# Autodesk Inventor assembly: maze_version2
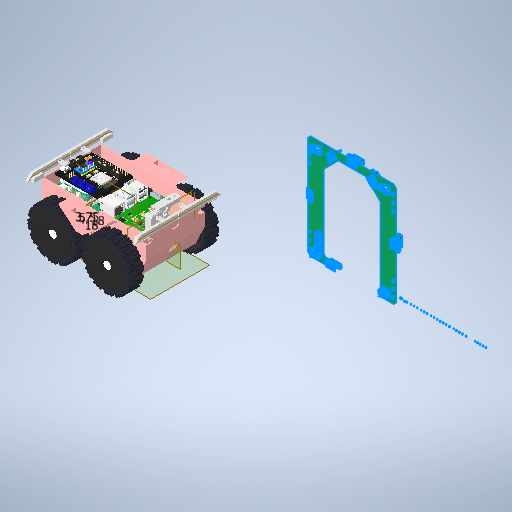
[picture p0: Inventor's stored thumbnail of the model, 512x512]
Saved by Autodesk Inventor 2025 (Build 290162000, 162)
## iProperties
Created: 2026-06-23
Part Number: maze_version2
Document SubType Name: Assembly
Designer: garin
Author: garin
## Documents named in this file (29)
- C:\Users\Leva\Documents\Git\TheseusV2_Maze\Construction\Theseus_v2\Theseus_v2.iam
- C:\Users\Leva\Documents\Git\TheseusV2_Maze\Construction\Theseus_v2\DDSM210.ipt
- C:\Users\Leva\Documents\Git\TheseusV2_Maze\Construction\akkum_TSE\akkum.iam
- C:\Users\Leva\Documents\Git\TheseusV2_Maze\Construction\Theseus_v2\low_part.ipt
- C:\Users\Leva\Documents\Git\TheseusV2_Maze\Construction\Theseus_v2\USBCamera.ipt
- C:\Users\Leva\Documents\Git\TheseusV2_Maze\Construction\maze_test_course\maze_test_course.ipt
- C:\Users\Leva\Documents\Git\TheseusV2_Maze\Construction\Theseus_v2\TCS34725.ipt
- C:\Users\Leva\Documents\Git\TheseusV2_Maze\Construction\Theseus_v2\optopar.ipt
- C:\Users\Leva\Documents\Git\TheseusV2_Maze\Construction\Theseus_v2\magasin.ipt
- C:\Users\Leva\Documents\Git\TheseusV2_Maze\Construction\Theseus_v2\LD19_v2.ipt
- C:\Users\Leva\Documents\Git\TheseusV2_Maze\Construction\Theseus_v2\sensor board.ipt
- C:\Users\Leva\Documents\Git\TheseusV2_Maze\Construction\Theseus_v2\VL53l1X.ipt
- C:\Users\Leva\Documents\Git\TheseusV2_Maze\Construction\Theseus_v2\mother_board\mb_mother_board.iam
- C:\Users\Leva\Documents\Git\TheseusV2_Maze\Construction\Theseus_v2\OCS-D008 B.ipt
- C:\Users\Leva\Documents\Git\TheseusV2_Maze\Construction\Theseus_v2\up_part.ipt
- C:\Users\Leva\Documents\Git\TheseusV2_Maze\Construction\Theseus_v2\Micro limit switch.ipt
- C:\Users\Leva\Documents\Git\TheseusV2_Maze\Construction\Theseus_v2\microswitch_cap.ipt
- C:\Users\Leva\Documents\Git\TheseusV2_Maze\Construction\Theseus_v2\Micro limit switch_MIR.ipt
- C:\Users\Leva\Documents\Git\TheseusV2_Maze\Construction\Theseus_v2\microswitch_cap_MIR.ipt
- C:\Users\Leva\Downloads\PLS-6R-D1\PLS-6R-D1.ipt
- C:\Users\Leva\Documents\Git\TheseusV2_Maze\Construction\Theseus_v2\Hafele_mini_latch.ipt
- C:\Users\Leva\Documents\Git\TheseusV2_Maze\Construction\Theseus_v2\power_board.ipt
- C:\Users\Leva\Documents\Git\TheseusV2_Maze\Construction\Theseus_v2\ihlp5050ceer2r2m01.ipt
- C:\Users\garin\Documents\models\altium_model\molex\mini_spox\0022057045\0022057045.ipt
- C:\Users\Leva\Documents\Git\TheseusV2_Maze\Construction\Theseus_v2\0022057045\0022057045.ipt
- C:\Users\garin\Documents\Git\TheseusV2_Maze\Schematic\TSE_power_control_board\m.ipt
- C:\Users\Leva\Documents\Git\TheseusV2_Maze\Schematic\TSE_power_control_board\TSE_power_control_board.ipt
- C:\Users\Leva\Documents\Git\TheseusV2_Maze\Construction\Theseus_v2\sensor_commutation_board\sensor_commutation_board.iam
- C:\Users\Leva\Documents\Git\TheseusV2_Maze\Schematic\TSE_sensor_commutation_board\TSE_sensor_commutation_board2.ipt
## Components (41 placed, 27 different names)
1. low_part:1 — Заподлицо:1, Заподлицо:2, Заподлицо:3, Совмещение:1, Совмещение:2, Совмещение:3, Совмещение:7, Совмещение:8, Совмещение:9, Совмещение:27, Совмещение:28, Совмещение:29, Совмещение:30, Совмещение:31, Совмещение:32, Совмещение:42, Совмещение:43, Совмещение:44, Совмещение:45, Совмещение:46, Совмещение:47, Совмещение:49, Угол:1, Совмещение:59, Совмещение:60, Совмещение:62, Совмещение:63, Заподлицо:14, Совмещение:64, Совмещение:65, Совмещение:66, Заподлицо:16, Заподлицо:17, Заподлицо:18, Совмещение:68, Совмещение:97, Совмещение:98, Совмещение:99, Совмещение:104, Совмещение:109, Совмещение:111, Совмещение:113, Совмещение:114, Совмещение:115, Совмещение:116, Совмещение:117, Совмещение:118, Заподлицо:29, Заподлицо:30
2. DDSM210:1 — Совмещение:27, Совмещение:28, Совмещение:29, Заподлицо:19
3. DDSM210:2 — Совмещение:1, Совмещение:2, Совмещение:3
4. DDSM210:3 — Совмещение:30, Совмещение:31, Совмещение:32
5. DDSM210:4 — Совмещение:7, Совмещение:8, Совмещение:9
6. akkum:2 [sub-assembly]
7. maze_test_course:1 — Совмещение:35
8. TCS34725:1 — Совмещение:45, Совмещение:46, Совмещение:47
9. optopar:1 — Совмещение:42, Совмещение:43, Совмещение:44
10. USBCamera:2 — Совмещение:49, Угол:1, Совмещение:68
11. magasin:1 — Совмещение:62, Совмещение:63, Заподлицо:14, Заподлицо:15
12. sensor board:1 — Заподлицо:9, Совмещение:54, Заподлицо:11, Совмещение:56, Угол:3, Совмещение:57, Совмещение:58, Совмещение:66, Заподлицо:16, Заподлицо:17, Совмещение:67, Совмещение:75, Заподлицо:20, Совмещение:76, Заподлицо:21, Совмещение:81, Совмещение:82, Заподлицо:22, Совмещение:83, Совмещение:84, Совмещение:91, Заподлицо:23, Заподлицо:26, Заподлицо:28
13. VL53l1X:1 — Заподлицо:9, Совмещение:54
14. VL53l1X:2 — Угол:3, Совмещение:57, Заподлицо:27, Заподлицо:28
15. VL53l1X:4 — Заподлицо:11, Совмещение:56, Совмещение:58
16. VL53l1X:5 — Совмещение:92, Заподлицо:24, Заподлицо:25, Заподлицо:26
17. mb_mother_board:1 [sub-assembly] — Совмещение:59, Совмещение:60, Совмещение:112, Совмещение:114
18. OCS-D008 B:1 — Заподлицо:15, Совмещение:64, Совмещение:65
19. up_part:1 — Совмещение:67, Заподлицо:18, Заподлицо:19, Совмещение:69, Совмещение:70, Совмещение:71, Совмещение:77, Совмещение:78, Совмещение:85, Совмещение:86, Совмещение:88, Совмещение:89
20. USBCamera:3 — Совмещение:69, Совмещение:70, Совмещение:71
21. USBCamera:4
22. Micro limit switch:1 — Совмещение:75, Заподлицо:20, Совмещение:76, Совмещение:79
23. microswitch_cap:1 — Совмещение:77, Совмещение:78, Совмещение:79
24. Micro limit switch_r:1 — Совмещение:80
25. microswitch_cap_r:1 — Совмещение:80
26. Micro limit switch:2 — Заподлицо:21, Совмещение:81, Совмещение:82, Совмещение:90
27. microswitch_cap:2 — Совмещение:88, Совмещение:89, Совмещение:90
28. Micro limit switch_r:2 — Заподлицо:22, Совмещение:83, Совмещение:84, Совмещение:87
29. microswitch_cap_r:2 — Совмещение:85, Совмещение:86, Совмещение:87
30. PLS-6R-D1:1 — Совмещение:91, Заподлицо:23, Совмещение:92, Заподлицо:24, Заподлицо:25
31. Hafele_mini_latch:1 — Совмещение:97, Совмещение:98, Совмещение:99
32. power_board:1 — Совмещение:100, Совмещение:101, Совмещение:104, Совмещение:106, Совмещение:108, Совмещение:110, Угол:4
33. ihlp5050ceer2r2m01:1 — Совмещение:100
34. ihlp5050ceer2r2m01:2 — Совмещение:101
35. 0022057045:1 — Совмещение:110, Угол:4
36. 0022057045:2 — Совмещение:106
37. m:1 — Совмещение:108, Совмещение:109
38. TSE_power_control_board:1 — Совмещение:115, Совмещение:116, Совмещение:117
39. sensor_commutation_board:1 [sub-assembly] — Совмещение:118, Заподлицо:29, Заподлицо:30
40. TSE_sensor_commutation_board2:1
41. LD19_v2:1 — Совмещение:111, Совмещение:112, Совмещение:113
## Relationships (97: Mate 72, Flush 22, Angle 3)
- Заподлицо:1 [Flush]: low_part:1
- Заподлицо:2 [Flush]: low_part:1
- Заподлицо:3 [Flush]: low_part:1
- Совмещение:1 [Mate]: low_part:1 ↔ DDSM210:2
- Совмещение:2 [Mate]: low_part:1 ↔ DDSM210:2
- Совмещение:3 [Mate]: low_part:1 ↔ DDSM210:2
- Совмещение:7 [Mate]: low_part:1 ↔ DDSM210:4
- Совмещение:8 [Mate]: low_part:1 ↔ DDSM210:4
- Совмещение:9 [Mate]: low_part:1 ↔ DDSM210:4
- Совмещение:27 [Mate]: low_part:1 ↔ DDSM210:1
- Совмещение:28 [Mate]: low_part:1 ↔ DDSM210:1
- Совмещение:29 [Mate]: low_part:1 ↔ DDSM210:1
- Совмещение:30 [Mate]: low_part:1 ↔ DDSM210:3
- Совмещение:31 [Mate]: low_part:1 ↔ DDSM210:3
- Совмещение:32 [Mate]: low_part:1 ↔ DDSM210:3
- Совмещение:35 [Mate]: maze_test_course:1
- Совмещение:42 [Mate]: low_part:1 ↔ optopar:1
- Совмещение:43 [Mate]: low_part:1 ↔ optopar:1
- Совмещение:44 [Mate]: low_part:1 ↔ optopar:1
- Совмещение:45 [Mate]: low_part:1 ↔ TCS34725:1
- Совмещение:46 [Mate]: low_part:1 ↔ TCS34725:1
- Совмещение:47 [Mate]: low_part:1 ↔ TCS34725:1
- Совмещение:49 [Mate]: low_part:1 ↔ USBCamera:2
- Угол:1 [Angle] (0 deg): low_part:1 ↔ USBCamera:2
- Заподлицо:9 [Flush]: sensor board:1 ↔ VL53l1X:1
- Совмещение:54 [Mate]: sensor board:1 ↔ VL53l1X:1
- Заподлицо:11 [Flush]: sensor board:1 ↔ VL53l1X:4
- Совмещение:56 [Mate]: sensor board:1 ↔ VL53l1X:4
- Угол:3 [Angle] (0 deg): sensor board:1 ↔ VL53l1X:2
- Совмещение:57 [Mate]: sensor board:1 ↔ VL53l1X:2
- Совмещение:58 [Mate] (3 mm): sensor board:1 ↔ VL53l1X:4
- Совмещение:59 [Mate]: low_part:1 ↔ mb_mother_board:1
- Совмещение:60 [Mate]: low_part:1 ↔ mb_mother_board:1
- Совмещение:62 [Mate] (0.2 mm): low_part:1 ↔ magasin:1
- Совмещение:63 [Mate] (0.2 mm): low_part:1 ↔ magasin:1
- Заподлицо:14 [Flush] (1.4 mm): low_part:1 ↔ magasin:1
- Заподлицо:15 [Flush] (-0.4 mm): magasin:1 ↔ OCS-D008 B:1
- Совмещение:64 [Mate] (0.5 mm): low_part:1 ↔ OCS-D008 B:1
- Совмещение:65 [Mate] (0.5 mm): low_part:1 ↔ OCS-D008 B:1
- Совмещение:66 [Mate]: low_part:1 ↔ sensor board:1
- Заподлицо:16 [Flush]: low_part:1 ↔ sensor board:1
- Заподлицо:17 [Flush]: low_part:1 ↔ sensor board:1
- Совмещение:67 [Mate]: sensor board:1 ↔ up_part:1
- Заподлицо:18 [Flush]: low_part:1 ↔ up_part:1
- Заподлицо:19 [Flush]: DDSM210:1 ↔ up_part:1
- Совмещение:68 [Mate]: low_part:1 ↔ USBCamera:2
- Совмещение:69 [Mate]: up_part:1 ↔ USBCamera:3
- Совмещение:70 [Mate] (0.5 mm): up_part:1 ↔ USBCamera:3
- Совмещение:71 [Mate] (0.5 mm): up_part:1 ↔ USBCamera:3
- Совмещение:75 [Mate]: sensor board:1 ↔ Micro limit switch:1
- Заподлицо:20 [Flush] (2.6 mm): sensor board:1 ↔ Micro limit switch:1
- Совмещение:76 [Mate] (-3 mm): sensor board:1 ↔ Micro limit switch:1
- Совмещение:77 [Mate] (0.25 mm): up_part:1 ↔ microswitch_cap:1
- Совмещение:78 [Mate] (0.2 mm): up_part:1 ↔ microswitch_cap:1
- Совмещение:79 [Mate]: Micro limit switch:1 ↔ microswitch_cap:1
- Совмещение:80 [Mate]: Micro limit switch_r:1 ↔ microswitch_cap_r:1
- Заподлицо:21 [Flush] (2.6 mm): sensor board:1 ↔ Micro limit switch:2
- Совмещение:81 [Mate]: sensor board:1 ↔ Micro limit switch:2
- Совмещение:82 [Mate] (-3 mm): sensor board:1 ↔ Micro limit switch:2
- Заподлицо:22 [Flush] (2.6 mm): sensor board:1 ↔ Micro limit switch_r:2
- Совмещение:83 [Mate]: sensor board:1 ↔ Micro limit switch_r:2
- Совмещение:84 [Mate] (-3 mm): sensor board:1 ↔ Micro limit switch_r:2
- Совмещение:85 [Mate] (0.25 mm): up_part:1 ↔ microswitch_cap_r:2
- Совмещение:86 [Mate] (0.2 mm): up_part:1 ↔ microswitch_cap_r:2
- Совмещение:87 [Mate]: Micro limit switch_r:2 ↔ microswitch_cap_r:2
- Совмещение:88 [Mate] (0.25 mm): up_part:1 ↔ microswitch_cap:2
- Совмещение:89 [Mate] (0.2 mm): up_part:1 ↔ microswitch_cap:2
- Совмещение:90 [Mate]: Micro limit switch:2 ↔ microswitch_cap:2
- Совмещение:91 [Mate]: sensor board:1 ↔ PLS-6R-D1:1
- Заподлицо:23 [Flush] (50 mm): sensor board:1 ↔ PLS-6R-D1:1
- Совмещение:92 [Mate]: VL53l1X:5 ↔ PLS-6R-D1:1
- Заподлицо:24 [Flush]: VL53l1X:5 ↔ PLS-6R-D1:1
- Заподлицо:25 [Flush]: VL53l1X:5 ↔ PLS-6R-D1:1
- Заподлицо:26 [Flush]: sensor board:1 ↔ VL53l1X:5
- Заподлицо:27 [Flush] (3 mm): VL53l1X:2
- Заподлицо:28 [Flush] (5 mm): sensor board:1 ↔ VL53l1X:2
- Совмещение:97 [Mate]: low_part:1 ↔ Hafele_mini_latch:1
- Совмещение:98 [Mate]: low_part:1 ↔ Hafele_mini_latch:1
- Совмещение:99 [Mate]: low_part:1 ↔ Hafele_mini_latch:1
- Совмещение:100 [Mate]: power_board:1 ↔ ihlp5050ceer2r2m01:1
- Совмещение:101 [Mate]: power_board:1 ↔ ihlp5050ceer2r2m01:2
- Совмещение:104 [Mate]: low_part:1 ↔ power_board:1
- Совмещение:106 [Mate]: power_board:1 ↔ 0022057045:2
- Совмещение:108 [Mate]: power_board:1 ↔ m:1
- Совмещение:109 [Mate] (10 mm): low_part:1 ↔ m:1
- Совмещение:110 [Mate]: power_board:1 ↔ 0022057045:1
- Угол:4 [Angle] (0 deg): power_board:1 ↔ 0022057045:1
- Совмещение:111 [Mate]: low_part:1 ↔ LD19_v2:1
- Совмещение:112 [Mate]: mb_mother_board:1 ↔ LD19_v2:1
- Совмещение:113 [Mate]: low_part:1 ↔ LD19_v2:1
- Совмещение:114 [Mate] (0.5 mm): low_part:1 ↔ mb_mother_board:1
- Совмещение:115 [Mate]: low_part:1 ↔ TSE_power_control_board:1
- Совмещение:116 [Mate]: low_part:1 ↔ TSE_power_control_board:1
- Совмещение:117 [Mate]: low_part:1 ↔ TSE_power_control_board:1
- Совмещение:118 [Mate]: low_part:1 ↔ sensor_commutation_board:1
- Заподлицо:29 [Flush]: low_part:1 ↔ sensor_commutation_board:1
- Заподлицо:30 [Flush]: low_part:1 ↔ sensor_commutation_board:1
